# Autodesk Inventor assembly: Control & Sense Head PCB Assm
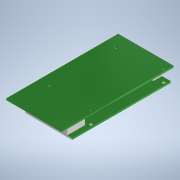
[picture p0: Inventor's stored thumbnail of the model, 180x180]
Saved by Autodesk Inventor 2021 (Build 250183000, 183)
## iProperties
Created: 2019-11-04
Part Number: Control & Sense Head PCB Assm
Document SubType Name: Assembly
Designer: jgray
Author: jgray
## Documents named in this file (3)
- M:\Printed Electronics\Gas Sensors\Prototypes\Prototype II -Cartridge Reader V3\Control & Sense Head PCB Assm.iam
- M:\Printed Electronics\Gas Sensors\Prototypes\Prototype II -Cartridge Reader V3\EVAL_ADICUP360.ipt
- M:\Printed Electronics\Gas Sensors\Prototypes\Prototype II -Cartridge Reader V3\PCB Control Board ADICUP1.ipt
## Components (2 placed, 2 different names)
1. EVAL_ADICUP360:1 — Mate:3, Mate:4, Mate:5
2. PCB Control Board ADICUP1:1 — Mate:3, Mate:4, Mate:5
## Relationships (3: Mate 3)
- Mate:3 (12 mm): EVAL_ADICUP360:1 ↔ PCB Control Board ADICUP1:1
- Mate:4: EVAL_ADICUP360:1 ↔ PCB Control Board ADICUP1:1
- Mate:5: EVAL_ADICUP360:1 ↔ PCB Control Board ADICUP1:1
